# Autodesk Inventor assembly: davinci_head_and_guide
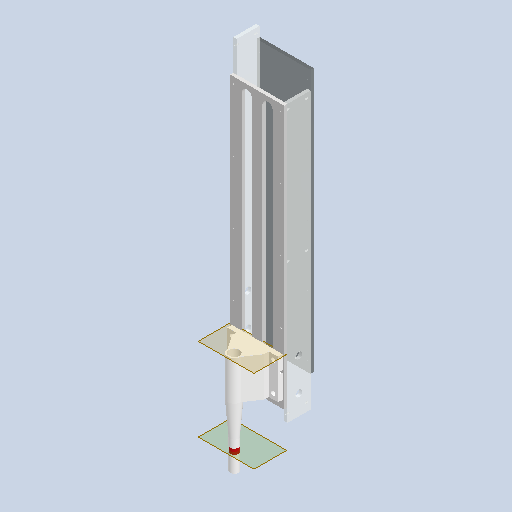
[picture p0: Inventor's stored thumbnail of the model, 512x512]
Saved by Autodesk Inventor 2022 (Build 260153000, 153)
## iProperties
Created: 2021-11-04
Part Number: davinci_head_and_guide
Document SubType Name: Assembly
Designer: espen
Author: espen
## Documents named in this file (5)
- C:\Users\alexw\Documents\Inventor\Projects\03_CurrentProjects\MasterThesis\PSM_V1_Rillenkugellager\Ueberarbeiteter DaVincikopf\davinci_head_and_guide.iam
- C:\Users\alexw\Documents\Inventor\Projects\03_CurrentProjects\MasterThesis\PSM_V1_Rillenkugellager\Slot profile.ipt
- C:\Users\alexw\Documents\Inventor\Projects\03_CurrentProjects\MasterThesis\PSM_V1_Rillenkugellager\Side plate profile.ipt
- C:\Users\alexw\Documents\Inventor\Projects\03_CurrentProjects\MasterThesis\PSM_V1_Rillenkugellager\Back plate profile.ipt
- C:\Users\alexw\Documents\Inventor\Projects\03_CurrentProjects\MasterThesis\PSM_V1_Rillenkugellager\Guide.ipt
## Components (5 placed, 4 different names)
1. Slot profile:1 — Fluchtend:6, Passend:11, Einfügen:1, Fluchtend:7
2. Side plate profile:1 — Fluchtend:3, Fluchtend:4
3. Side plate profile:2 — Mate:10, Fluchtend:6, Passend:11, Fluchtend:7
4. Back plate profile:1 — Mate:10, Fluchtend:3, Fluchtend:4
5. Guide:1 — Einfügen:1
## Relationships (7: Flush 4, Mate 2, Insert 1)
- Mate:10: Side plate profile:2 ↔ Back plate profile:1
- Fluchtend:3 [Flush]: Side plate profile:1 ↔ Back plate profile:1
- Fluchtend:4 [Flush]: Side plate profile:1 ↔ Back plate profile:1
- Fluchtend:6 [Flush]: Slot profile:1 ↔ Side plate profile:2
- Passend:11 [Mate]: Slot profile:1 ↔ Side plate profile:2
- Einfügen:1 [Insert]: Slot profile:1 ↔ Guide:1
- Fluchtend:7 [Flush]: Slot profile:1 ↔ Side plate profile:2
